# Autodesk Inventor assembly: Evaporator
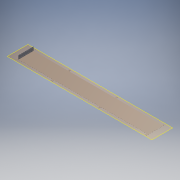
[picture p0: Inventor's stored thumbnail of the model, 180x180]
Saved by Autodesk Inventor 2016 (Build 200138000, 138)
## iProperties
Created: 2017-06-28
Part Number: Evaporator
Document SubType Name: Assembly
Designer: Roeder
Author: Roeder
## Documents named in this file (3)
- T:\07 Projects\2017\Gen3 Indis\01_Documents\Evaporator Specification\Model\Evaporator.iam
- T:\07 Projects\2017\Gen3 Indis\01_Documents\Evaporator Specification\Model\Parts\Baseplate.ipt
- T:\07 Projects\2017\Gen3 Indis\01_Documents\Evaporator Specification\Model\Parts\Cover Plate.ipt
## Components (2 placed, 2 different names)
1. Baseplate:1 — Flush:1, Flush:2
2. Cover Plate:1 — Flush:1, Flush:2
## Relationships (2: Flush 2)
- Flush:1: Baseplate:1 ↔ Cover Plate:1
- Flush:2: Baseplate:1 ↔ Cover Plate:1
